# Autodesk Inventor assembly: NewSmallSize(2xl)
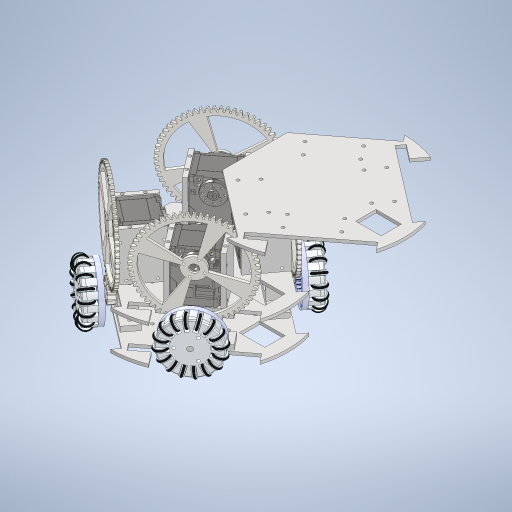
[picture p0: Inventor's stored thumbnail of the model, 512x512]
Saved by Autodesk Inventor 2023 (Build 270158000, 158)
## iProperties
Created: 2022-09-27
Part Number: NewSmallSize(2xl)
Document SubType Name: Assembly
Designer: hiago.sodre
Author: hiago.sodre
## Documents named in this file (5)
- C:\Users\hiago.sodre\Downloads\ssl_CAD-main\Model_2XL430-W250-T\NewSmallSize(2xl).iam
- C:\Users\hiago.sodre\Downloads\ssl_CAD-main\Model_2XL430-W250-T\newbase.ipt
- C:\Users\hiago.sodre\Downloads\ssl_CAD-main\Model_2XL430-W250-T\soporte_eje_omni.ipt
- C:\Users\hiago.sodre\Downloads\ssl_CAD-main\Model_2XL430-W250-T\EjeRueda.iam
- C:\Users\hiago.sodre\Downloads\ssl_CAD-main\Model_2XL430-W250-T\2XL-430montado.iam
## Components (15 placed, 4 different names)
1. newbase:1 — Mate:2, Mate:3, Mate:6, Mate:7, Mate:9, Mate:10, Mate:12, Mate:13
2. newbase:2 — Mate:16, Mate:17
3. newbase:3
4. soporte_eje_omni:1 — Mate:2, Mate:3, De rotación:1
5. soporte_eje_omni:2 — Mate:6, Mate:7, Mate:8
6. EjeRueda:1 [sub-assembly] — Mate:8
7. EjeRueda:2 [sub-assembly] — De rotación:1
8. EjeRueda:3 [sub-assembly] — Mate:15
9. EjeRueda:4 [sub-assembly] — Mate:11
10. soporte_eje_omni:5 — Mate:9, Mate:10, Mate:11, Mate:16, Mate:17
11. soporte_eje_omni:6 — Mate:12, Mate:13, Mate:15
12. 2XL-430montado:1 [sub-assembly]
13. 2XL-430montado:2 [sub-assembly]
14. 2XL-430montado:3 [sub-assembly]
15. 2XL-430montado:4 [sub-assembly]
## Relationships (14: Mate 13, RevoluteJoint 1)
- Mate:2: newbase:1 ↔ soporte_eje_omni:1
- Mate:3: newbase:1 ↔ soporte_eje_omni:1
- Mate:6: newbase:1 ↔ soporte_eje_omni:2
- Mate:7: newbase:1 ↔ soporte_eje_omni:2
- Mate:8: soporte_eje_omni:2 ↔ EjeRueda:1
- Mate:9: newbase:1 ↔ soporte_eje_omni:5
- Mate:10: newbase:1 ↔ soporte_eje_omni:5
- Mate:11: EjeRueda:4 ↔ soporte_eje_omni:5
- Mate:12: newbase:1 ↔ soporte_eje_omni:6
- Mate:13: newbase:1 ↔ soporte_eje_omni:6
- Mate:15: EjeRueda:3 ↔ soporte_eje_omni:6
- Mate:16: newbase:2 ↔ soporte_eje_omni:5
- Mate:17: newbase:2 ↔ soporte_eje_omni:5
- De rotación:1 [RevoluteJoint]: soporte_eje_omni:1 ↔ EjeRueda:2
